# Autodesk Inventor assembly: motor_assembly
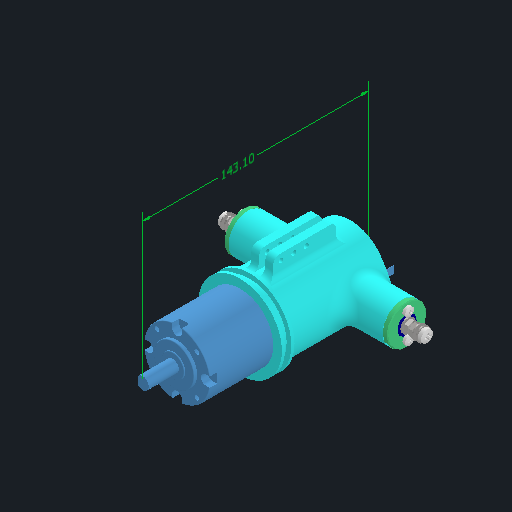
[picture p0: Inventor's stored thumbnail of the model, 512x512]
Saved by Autodesk Inventor 2024 (Build 280153000, 153)
## iProperties
Created: 2023-04-15
Part Number: motor_assembly
Document SubType Name: Assembly
Designer: user
Author: user
## Documents named in this file (4)
- D:\Docs\Robot\3d\motor_assembly\midel\motor_assembly_M.iam
- D:\Docs\Robot\3d\default_components\motor.ipt
- D:\Docs\Robot\3d\motor_assembly\midel\lower_arm.ipt
- D:\Docs\Robot\3d\motor_assembly\bushing_assembly\bushing_assembly.iam
## Components (4 placed, 3 different names)
1. motor:1 — Совмещение:1, Совмещение:2, Совмещение:3, Заподлицо:1
2. lower_arm:1 — Заподлицо:1, Совмещение:4, Вставка:1, Вставка:2
3. bushing_assembly:1 [sub-assembly] — Вставка:1
4. bushing_assembly:2 [sub-assembly] — Вставка:2
## Relationships (7: Mate 4, Insert 2, Flush 1)
- Совмещение:1 [Mate]: motor:1
- Совмещение:2 [Mate]: motor:1
- Совмещение:3 [Mate]: motor:1
- Заподлицо:1 [Flush]: motor:1 ↔ lower_arm:1
- Совмещение:4 [Mate]: lower_arm:1
- Вставка:1 [Insert]: lower_arm:1 ↔ bushing_assembly:1
- Вставка:2 [Insert]: lower_arm:1 ↔ bushing_assembly:2
